# Autodesk Inventor assembly: Assembly_HoliSheet_v6
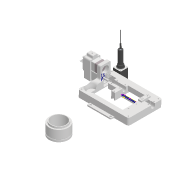
[picture p0: Inventor's stored thumbnail of the model, 180x180]
Saved by Autodesk Inventor 2022 (Build 260153000, 153)
## iProperties
Created: 2023-01-07
Part Number: Assembly_HoliSheet_v6
Document SubType Name: Assembly
Designer: diederichbenedict
Author: diederichbenedict
## Documents named in this file (10)
- C:\Users\diederichbenedict\Dropbox\Dokumente\Promotion\PROJECTS\HoLiSheet\INVENTOR\Assembly_HoliSheet_v6.iam
- C:\Users\diederichbenedict\Dropbox\Dokumente\Promotion\PROJECTS\HoLiSheet\INVENTOR\Assemlby_Scanner_v1.iam
- C:\Users\diederichbenedict\Dropbox\Dokumente\Promotion\PROJECTS\HoLiSheet\INVENTOR\11_Wellplatespacer.ipt
- C:\Users\diederichbenedict\Dropbox\Dokumente\Promotion\PROJECTS\HoLiSheet\INVENTOR\00_microscope_turret.ipt
- C:\Users\diederichbenedict\Dropbox\Dokumente\Promotion\PROJECTS\HoLiSheet\INVENTOR\00_NEMA8.ipt
- C:\Users\diederichbenedict\Dropbox\Dokumente\Promotion\PROJECTS\HoLiSheet\INVENTOR\00_Joy-IT-B20SHD4353_NEMA8_captive.ipt
- C:\Users\diederichbenedict\Dropbox\Dokumente\Promotion\PROJECTS\HoLiSheet\INVENTOR\Holisheet_NEMA8_connector.ipt
- C:\Users\diederichbenedict\Dropbox\Dokumente\Promotion\PROJECTS\HoLiSheet\INVENTOR\Holisheet_NEMA8_Syringe_pusher.ipt
- C:\Users\diederichbenedict\Dropbox\Dokumente\Promotion\PROJECTS\HoLiSheet\INVENTOR\10_Wellplate_base_v6.ipt
- C:\Users\diederichbenedict\Dropbox\Dokumente\Promotion\PROJECTS\HoLiSheet\INVENTOR\Holisheet_tubeclamp.ipt
## Components (11 placed, 9 different names)
1. 10_Wellplate_base_v6:1 — Passend:2, Winkel:1, Einfügen:1, Winkel:2, Fluchtend:1, Fluchtend:2, Einfügen:2, Winkel:3, Fluchtend:8, Fluchtend:9, Fluchtend:10
2. Assemlby_Scanner_v1:1 [sub-assembly] — Passend:2, Winkel:1, Fluchtend:1, Fluchtend:2
3. 11_Wellplatespacer:1 — Einfügen:1, Winkel:2
4. 00_microscope_turret:1
5. 00_NEMA8:1 — Einfügen:2, Winkel:3, Passend:4, Fluchtend:4, Fluchtend:5, Fluchtend:6
6. 00_Joy-IT-B20SHD4353_NEMA8_captive:1
7. 00_NEMA8:2 — Passend:4, Fluchtend:4, Fluchtend:5, Fluchtend:7
8. Holisheet_NEMA8_connector:1 — Fluchtend:6
9. Holisheet_NEMA8_Syringe_pusher:1 — Fluchtend:7
10. Holisheet_tubeclamp:1 — Fluchtend:8, Fluchtend:9, Fluchtend:10
11. Holisheet_tubeclamp:2
## Relationships (16: Flush 9, Angle 3, Mate 2, Insert 2)
- Passend:2 [Mate] (1.4 mm): 10_Wellplate_base_v6:1 ↔ Assemlby_Scanner_v1:1
- Winkel:1 [Angle] (0 deg): 10_Wellplate_base_v6:1 ↔ Assemlby_Scanner_v1:1
- Einfügen:1 [Insert]: 10_Wellplate_base_v6:1 ↔ 11_Wellplatespacer:1
- Winkel:2 [Angle] (180 deg): 10_Wellplate_base_v6:1 ↔ 11_Wellplatespacer:1
- Fluchtend:1 [Flush]: 10_Wellplate_base_v6:1 ↔ Assemlby_Scanner_v1:1
- Fluchtend:2 [Flush]: 10_Wellplate_base_v6:1 ↔ Assemlby_Scanner_v1:1
- Einfügen:2 [Insert]: 10_Wellplate_base_v6:1 ↔ 00_NEMA8:1
- Winkel:3 [Angle] (180 deg): 10_Wellplate_base_v6:1 ↔ 00_NEMA8:1
- Passend:4 [Mate] (0.5 mm): 00_NEMA8:1 ↔ 00_NEMA8:2
- Fluchtend:4 [Flush]: 00_NEMA8:1 ↔ 00_NEMA8:2
- Fluchtend:5 [Flush]: 00_NEMA8:1 ↔ 00_NEMA8:2
- Fluchtend:6 [Flush]: 00_NEMA8:1 ↔ Holisheet_NEMA8_connector:1
- Fluchtend:7 [Flush]: 00_NEMA8:2 ↔ Holisheet_NEMA8_Syringe_pusher:1
- Fluchtend:8 [Flush]: 10_Wellplate_base_v6:1 ↔ Holisheet_tubeclamp:1
- Fluchtend:9 [Flush]: 10_Wellplate_base_v6:1 ↔ Holisheet_tubeclamp:1
- Fluchtend:10 [Flush]: 10_Wellplate_base_v6:1 ↔ Holisheet_tubeclamp:1
